# Autodesk Inventor assembly: 043-DXP
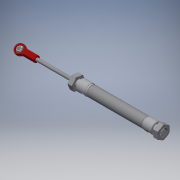
[picture p0: Inventor's stored thumbnail of the model, 180x180]
Saved by Autodesk Inventor 2019.4 (Build 234330000, 330)
## iProperties
Category: PARTsolutions
Company: BIMBA
Created: 2019-03-16
Part Number: 043-DXP
Catalog Web Link: www.cadenas.de
Description: Original Line Standard Air Cylinders-Standard Air Cylinders
Vendor: BIMBA
Document SubType Name: Assembly
Designer: psadmin
Manufacturer: BIMBA
Mass: 39.6638 g
Surface Area: 302.251 cm^2
Volume: 39.6638 cm^3
Density: 1 g/cm^3
PSOL_IDENT_0: {$CADENAS_DATA\23d-libs\bimba\bimba\bimba_imperial\bimba_full_line\original_line_cylinders\standard_
PSOL_IDENT_1: air_cylinders\standard_air_cylinder_asmtab.prj},322 {VTYP=3D},{STYP=ASSTAB},{NB=043-DXP},{LINA=043-D
PSOL_IDENT_2: XP},{NN=Original Line Standard Air Cylinders},{DATE=05.03.2019 14:21:37},{GEOMDATE=15.02.2019 06:55:
PSOL_IDENT_3: 59},{VERSION=},{LINEID=50},{WBVAR=STROKE,ACTING,MNT,DER,NR,BM,CO,OO,VO,M,EE,EEL,K,Q,Y,G,T,HL,B,H,SER
PSOL_IDENT_4: ,SR,NT,W,STPT1,STPT2,STPT3,STPT4,MB,PB,PRC,TB,MN},{WBNUMERIC=STROKE,EEL}  {NB=043-DXP},{LINA=043-DXP
PSOL_IDENT_5: },{KT=DUMMY},{PN=043-DXP},{PNC=043-DXP},{PNA=(NO ACCESSORIES)},{DASH=-},{BORE1=0.75000000},{BORE=3/4
PSOL_IDENT_6: \" (04)},{BOREPN=04},{STROKE=3.000},{STROKEALG=[0.011:50/0.001]},{STROKE1=3.000},{ACTING=D},{ACTINGA
PSOL_IDENT_7: LG= '' , 'Single Acting (SA)' , 'R' , 'Reverse Single Acting (SA)' , 'D' , 'Double Acting (SA)' },{A
PSOL_IDENT_8: CTINGPN=D},{MNT=XP},{MNTALG= '' , 'Front Nose Mounting (SA)' , 'P' , 'Rear Pivot Mounting (SA)' , 'X
PSOL_IDENT_9: P' , 'Double End or Pivot Mounting (SA)' , 'X' , 'Double End Mounting (SA)' , 'BF' , 'Front Block Mo
PSOL_IDENT_10: unting (SA)' , 'BR' , 'Rear Block Mounting for Vertical Positioning (SA)' , 'BFT' , 'Front Block Tru
PSOL_IDENT_11: nnion Mounting (SA)' , 'BRT' , 'Rear Block Trunnion Mounting (SA)' },{TYPE=},{MNTPN=XP},{DER=},{DERA
PSOL_IDENT_12: LG= '' , 'N/A' },{NR=},{NRALG= '' , 'N/A' },{NRPN=},{BM=},{BMALG= '' , 'N/A' },{BMPN=},{CO=},{COALG=
PSOL_IDENT_13: '' , 'N/A' },{OO=},{OOALG= '', 'N/A' },{OOPN=},{VO=Z},{VOALG= 'Z' , 'N/A' },{VOPN=},{OOVOPN=},{M=},
PSOL_IDENT_14: {MALG= '', 'Without Magnet', 'M', 'With Magnet' },{EE=},{EEL=0.000},{EEMAX=47.0000},{EEALG= '', 'Wit
PSOL_IDENT_15: hout Extra Extension', 'EE', 'With Extra Extension' },{EELALG=0},{EEPN=},{EEPN1=0.000},{K=},{KALG= ''
PSOL_IDENT_16: , 'Standard' , 'K' , 'Ports Rotated 90deg K' },{KPN=},{Q=},{QALG= '' , 'N/A' },{QPN=},{Y=},{YALG= ''
PSOL_IDENT_17: , 'Without Pivot Bushing' , 'Y' , 'With Pivot Bushing' },{YPN=},{YCON=},{F=},{FALG= '', 'Non-Coated
PSOL_IDENT_18: (Standard)', 'F', 'Molycoated' },{FPN=},{G=},{GPN=},{GPN99=},{T=},{TALG= '' , 'Standard -20° to 200
PSOL_IDENT_19: °F (-29° to 95°C)' , 'N' , 'Low Temperature' , 'V' , 'High Temperature' },{NPN=},{VPN=},{HL=},{HLALG=
PSOL_IDENT_20: '' , 'Without Low Pressure Hydraulic' , 'HL' , 'With Low Pressure Hydraulic' },{B=},{BALG= '', 'W/o
PSOL_IDENT_21: ut Bumpers' , 'B' , 'W/ Bumpers' },{BPN=},{H=},{HALG= '', 'N/A' },{HPN=},{SER=},{SERALG= '' , 'Witho
PSOL_IDENT_22: ut Spring Extend/Return' , 'JS' , 'With Spring Return' , 'JR' , 'With Spring Extend' },{SR=},{SRALG=
PSOL_IDENT_23: '' , 'Standard Stainless Steel' },{SRPN=},{SRCON=0},{NT=},{NTPN=},{W=},{WALG= '' , 'Without Wiper'
PSOL_IDENT_24: , 'W' , 'With Wiper' },{WPN=},{E=},{EALG= '' , 'Standard Seals/Lube' , 'E' , 'Non-Lube Seals/Lube' }
PSOL_IDENT_25: ,{EPN=},{ST=},{STALG= '' , 'N/A' },{STPT1=},{STPT1ALG= '' , 'N/A' },{STPT2=},{STPT2ALG= '' , 'N/A' }
PSOL_IDENT_26: ,{STPT3=},{STPT3ALG= '' , 'N/A' },{STPT4=},{STPT4ALG= '' , 'N/A' },{STPN=},{MB=},{MBALG= '' , 'Witho
PSOL_IDENT_27: ut Mounting Bracket' , 'F,D-129' , 'D-129 (front)'  , 'R,D-129' , 'D-129 (rear)' , '2x,D-129' , 'D-1
PSOL_IDENT_28: 29 (front & rear)'},{MBPN=},{MBPNALL=D-129},{MBPNALLREAR=D-129},{PB=},{PBALG= '' , 'Without Pivot Br
PSOL_IDENT_29: acket' , 'D-13498-A' , 'D-13498-A' },{PBPN=},{PBPNALL=D-13498-A},{PRC=},{PRCALG= '' , 'W/out Pivot R
PSOL_IDENT_30: od Clevis' , 'F,D-166-3' , 'D-166-3 (front)' },{PRCPN=},{PRCPNALL=D-166-3},{TB=},{TBALG= '' , 'N/A'
PSOL_IDENT_31: },{TBPN=},{TBPNALL=},{MN=},{MNALG= '' , 'N/A' },{MNPN=},{MNCONF=},{MNCONR=},{TLEN=4.2555},{FRAC=14.7
PSOL_IDENT_32: 500},{RGCON=},{RGDACCON=R},{RHCON=P},{RHCON1=P},{RHCONON=1},{RHACCON=},{FNUTCON=1},{RNUTCON=1},{FNUT
PSOL_IDENT_33: PN=D-9},{RNUTPN=D-9},{FNUTTRANS=0.0000},{RNUTTRANS=0.0000},{VHOLECON=0},{A1=1.5940},{A1N=0.8750},{A1
PSOL_IDENT_34: P=1.5940},{A1B=1.5940},{A4=0.2525},{A4N=0.3130},{A4P=0.2525},{A5=0.0300},{A1H=1.594},{A1NH=0.5310},{
PSOL_IDENT_35: A1PH=1.5940},{A1BH=1.0940},{A1SH=1.2190},{A2H=0.2190},{A2NH=0.2190},{LENGTH=3.7500},{LENGTH1=3.7500}
PSOL_IDENT_36: ,{LENGTH2=3.8100},{MUL=3.0000},{MUL11=3.0000},{MUL22=8.07},{MUL33=5.0700},{MUL2=3.0000},{MUL211=3.00
PSOL_IDENT_37: 00},{MUL222=2.6900},{MUL233=1.6900},{SSS=6.0000},{RGLEN=1.3715},{RHLEN=1.1230},{SSS1=4.0000},{A13=1.
PSOL_IDENT_38: 3120},{DIF=0.0000},{G5=0.6250},{ON=0},{SSADD=0.0000},{BADD=0.0000},{MADD=0.0000},{NVADD=0.0000},{TRA
PSOL_IDENT_39: CKL=3.9655},{TRACKCON=D-74168},{TRIMCON=0},{TRIMCON1=0},{PINCON=D-51},{FSPACE=0.7140},{SPACE=0.0750}
PSOL_IDENT_40: ,{TEXT=0.1312},{S1=1.0000},{D1=0.8325},{D1N=0.8050},{D1B=0.8625},{D1P=0.8325},{FA=0.940},{RA=0.9400}
PSOL_IDENT_41: ,{PPATH=standard_air_cylinder_asmtpl.prj},{MATALGHTML=<b>Standard Original Line:</b><dl><dt>Rod:</dt
PSOL_IDENT_42: ><dd>- Stainless Steel</dd><dd>&nbsp;&nbsp;(5/16 9/16 Bores)</dd><dd>- High Strength Carbon Steel</d
PSOL_IDENT_43: d><dd>&nbsp;&nbsp;(3/4 3 Bore)</dd><dd>- Stainless Steel</dd><dd>&nbsp;&nbsp;(X style DXP/DX/DXDE)</
PSOL_IDENT_44: dd><dt>Bearings:</dt><dd>- Sintered Bronze</dd><dt>Body:</dt><dd>- 304 Stainless Steel</dd><dt>End C
PSOL_IDENT_45: aps:</dt><dd>- Aluminum</dd><dt>Seals:</dt><dd>- Buna N</dd></dl>},{ASSCFGPRA=04DXP},{MBPNA=},{MNPNA=
PSOL_IDENT_46: },{PRCPNA=},{ASSOPTACC=STPT4},{A=6.75},{HADD=0.0000},{WFL=0.25},{QADD=0.000},{QADD1=0.440},{TEST=3.0
PSOL_IDENT_47: 000},{MNTB=},{STDNUTF=1},{STDNUTR=1},{STRK2D=0},{X2D=2},{STROKESW=3.000},{EESW=0.000},{FCD=0},{BCD=0
PSOL_IDENT_48: },{RCD=0},{CUSTADD=2.000},{FT=1/4-28 UNF-2A},{FT1=1/4-28 UNF-2A},{FT2=5/8-18 UNF-2A},{PORT=1/8 NPT},
PSOL_IDENT_49: {FT11=1/2-20 UNF-2A},{FT12=5/8-18 UNF-2A},{B1=}
NN: Original Line Standard Air Cylinders
NT: Standard Male Thread
NB: 043-DXP
NBSYN: $PNC.
LINA: 043-DXP
PN: 043-DXP
PNA: (NO ACCESSORIES)
BORE: 3/4" (04)
STROKE: 3
ACTING: Double [D]
MNT: Universal Double End or Rear Pivot [XP]
DER: N/A
NR: N/A
BM: N/A
CO: N/A
OO: N/A
VO: N/A
M: Without Magnet Piston
EE: Standard Rod Extension
EEL: 0
K: Standard
Q: N/A
Y: Standard Pivot Style
G: Standard Grease Lube
T: Standard -20° to 200°F (-29° to 95°C)
HL: Standard 250 PSI Air
B: Without Bumpers
H: N/A
SER: Without Failsafe Spring Extend/Return
SR: Standard Stainless Steel
W: Without Wiper
STPT1: N/A
STPT2: N/A
STPT3: N/A
STPT4: N/A
MB: Without Mounting Bracket
PB: Without Pivot Bracket
PRC: Without Piston Rod Clevis
TB: N/A
MN: N/A
A: 6.75
SUPPLIER: BIMBA
ARTICLENO: 043-DXP
BOMINFO: 043-DXP
CREATOR: CADENAS GmbH
Title: 043-DXP
Author: Cadenas PARTsolutions
Comments: Standard Air Cylinders
## Documents named in this file (7)
- T:\EIT\2020 Infinite Recharge\2020 ROBOT\COMMON PARTS\AIR CYLINDERS\043-DXP\AIS2019\043-DXP.iam
- T:\EIT\2020 Infinite Recharge\2020 ROBOT\COMMON PARTS\AIR CYLINDERS\043-DXP\AIS2019\043-DXP0000000_0_dummy.ipt
- T:\EIT\2020 Infinite Recharge\2020 ROBOT\COMMON PARTS\AIR CYLINDERS\043-DXP\AIS2019\04R000-0_rod_guide.ipt
- T:\EIT\2020 Infinite Recharge\2020 ROBOT\COMMON PARTS\AIR CYLINDERS\043-DXP\AIS2019\04R-4_25550.ipt
- T:\EIT\2020 Infinite Recharge\2020 ROBOT\COMMON PARTS\AIR CYLINDERS\043-DXP\AIS2019\04P0000_rear_head.ipt
- T:\EIT\2020 Infinite Recharge\2020 ROBOT\COMMON PARTS\AIR CYLINDERS\043-DXP\AIS2019\043-DXP0000_rod.ipt
- T:\EIT\2020 Infinite Recharge\2020 ROBOT\COMMON PARTS\AIR CYLINDERS\TieRod End\60685K321_PTFE-LINED ALUMINUM BALL JOINT ROD END.ipt
## Components (6 placed, 6 different names)
1. 043-DXP0000000_0_dummy:1
2. 04R000-0_rod_guide:1 — Insert:1, Insert:2, Angle:1
3. 04R-4_25550:1 — Insert:2, Insert:3
4. 04P0000_rear_head:1 — Insert:3, Angle:1, Angle:2
5. 043-DXP0000_rod:1 — Insert:1, Insert:6
6. 60685K321_PTFE-LINED ALUMINUM BALL JOINT ROD END:1 — Insert:6, Angle:2
## Relationships (6: Insert 4, Angle 2)
- Insert:1: 04R000-0_rod_guide:1 ↔ 043-DXP0000_rod:1
- Insert:2: 04R000-0_rod_guide:1 ↔ 04R-4_25550:1
- Insert:3: 04R-4_25550:1 ↔ 04P0000_rear_head:1
- Angle:1 (0 deg): 04R000-0_rod_guide:1 ↔ 04P0000_rear_head:1
- Insert:6: 043-DXP0000_rod:1 ↔ 60685K321_PTFE-LINED ALUMINUM BALL JOINT ROD END:1
- Angle:2 (0 deg): 04P0000_rear_head:1 ↔ 60685K321_PTFE-LINED ALUMINUM BALL JOINT ROD END:1
